# Autodesk Inventor assembly: Коробка передач в сборе
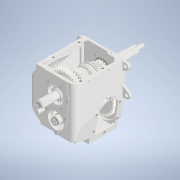
[picture p0: Inventor's stored thumbnail of the model, 180x180]
Saved by Autodesk Inventor 2021 (Build 250183000, 183)
## iProperties
Created: 2021-04-16
Part Number: Коробка передач в сборе
Document SubType Name: Assembly
Designer: Данил
Author: Данил
## Documents named in this file (9)
- C:\Users\Данил\Desktop\Коробка передач\Детали\Коробка передач в сборе.iam
- C:\Users\Данил\Desktop\Коробка передач\Детали\66-67. Картер коробки передач.ipt
- C:\Users\Данил\Desktop\Коробка передач\Детали\73. Вал вторичный в сборе.iam
- C:\Users\Данил\Desktop\Коробка передач\Детали\69. Блок шестерен промежуточного вала.iam
- C:\Users\Данил\Desktop\Коробка передач\Детали\74. Вал первичный в сборе.iam
- C:\Users\Данил\Desktop\Коробка передач\Детали\71. Блок шестерен заднего хода.iam
- C:\Users\Данил\Desktop\Коробка передач\Детали\74. Ось блока заднего хода.ipt
- C:\Users\Данил\Desktop\Коробка передач\Детали\73. Крышка подшипника.ipt
- C:\Users\Данил\Desktop\Коробка передач\Детали\75. Прокладка крышки.ipt
## Components (8 placed, 8 different names)
1. 66-67. Картер коробки передач:1 — Совмещение:1, Совмещение:2, Совмещение:3, Совмещение:4, Совмещение:6, Совмещение:7, Совмещение:8, Совмещение:9, Совмещение:10
2. 74. Вал первичный в сборе:1 [sub-assembly] — Совмещение:1, Совмещение:11
3. 73. Вал вторичный в сборе:1 [sub-assembly] — Совмещение:2
4. 69. Блок шестерен промежуточного вала:1 [sub-assembly] — Совмещение:3
5. 71. Блок шестерен заднего хода:1 [sub-assembly] — Совмещение:5
6. 74. Ось блока заднего хода:1 — Совмещение:4, Совмещение:5
7. 73. Крышка подшипника:1 — Совмещение:9, Совмещение:10, Совмещение:12
8. 75. Прокладка крышки:1 — Совмещение:6, Совмещение:7, Совмещение:8, Совмещение:11, Совмещение:12
## Relationships (12: Mate 12)
- Совмещение:1 [Mate]: 66-67. Картер коробки передач:1 ↔ 74. Вал первичный в сборе:1
- Совмещение:2 [Mate]: 66-67. Картер коробки передач:1 ↔ 73. Вал вторичный в сборе:1
- Совмещение:3 [Mate]: 66-67. Картер коробки передач:1 ↔ 69. Блок шестерен промежуточного вала:1
- Совмещение:4 [Mate]: 66-67. Картер коробки передач:1 ↔ 74. Ось блока заднего хода:1
- Совмещение:5 [Mate]: 71. Блок шестерен заднего хода:1 ↔ 74. Ось блока заднего хода:1
- Совмещение:6 [Mate]: 66-67. Картер коробки передач:1 ↔ 75. Прокладка крышки:1
- Совмещение:7 [Mate]: 66-67. Картер коробки передач:1 ↔ 75. Прокладка крышки:1
- Совмещение:8 [Mate]: 66-67. Картер коробки передач:1 ↔ 75. Прокладка крышки:1
- Совмещение:9 [Mate]: 66-67. Картер коробки передач:1 ↔ 73. Крышка подшипника:1
- Совмещение:10 [Mate]: 66-67. Картер коробки передач:1 ↔ 73. Крышка подшипника:1
- Совмещение:11 [Mate]: 74. Вал первичный в сборе:1 ↔ 75. Прокладка крышки:1
- Совмещение:12 [Mate]: 73. Крышка подшипника:1 ↔ 75. Прокладка крышки:1
